# Autodesk Inventor assembly: mt32_case
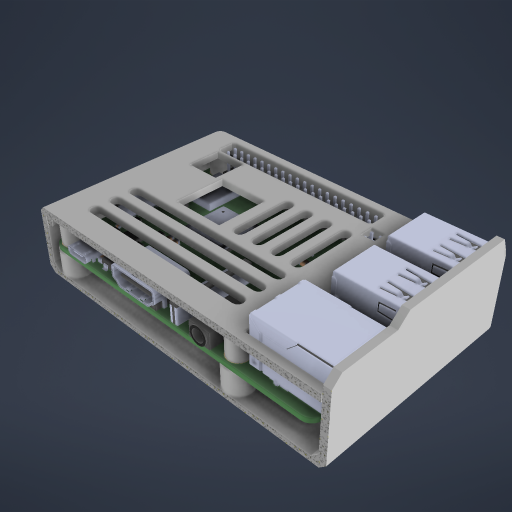
[picture p0: Inventor's stored thumbnail of the model, 512x512]
Saved by Autodesk Inventor 2024 (Build 280153000, 153)
## iProperties
Created: 2023-05-01
Part Number: mt32_case
Document SubType Name: Assembly
Designer: ancher
Author: ancher
## Documents named in this file (5)
- E:\RC\print_3d\mister\mt32_case\mt32_case.iam
- E:\RC\print_3d\mister\mt32_case\raspberry_pi3_b.ipt
- E:\RC\print_3d\mister\mt32_case\case_bottom.ipt
- E:\RC\print_3d\mister\mt32_case\case_top.ipt
- E:\RC\print_3d\mister\mt32_case\raspberry_pi3_b_.ipt
## Components (4 placed, 4 different names)
1. raspberry_pi3_b:1 — Mate:4, Mate:5, Mate:6, Mate:7, Mate:9
2. raspberry_pi3_b+:1 — Mate:10, Mate:11, Mate:12
3. case_bottom:1 — Mate:4, Mate:5, Mate:6, Mate:8, Mate:10, Mate:11, Mate:12
4. case_top:1 — Mate:7, Mate:8, Mate:9
## Relationships (9: Mate 9)
- Mate:4: raspberry_pi3_b:1 ↔ case_bottom:1
- Mate:5: raspberry_pi3_b:1 ↔ case_bottom:1
- Mate:6: raspberry_pi3_b:1 ↔ case_bottom:1
- Mate:7: raspberry_pi3_b:1 ↔ case_top:1
- Mate:8: case_bottom:1 ↔ case_top:1
- Mate:9: raspberry_pi3_b:1 ↔ case_top:1
- Mate:10: raspberry_pi3_b+:1 ↔ case_bottom:1
- Mate:11: raspberry_pi3_b+:1 ↔ case_bottom:1
- Mate:12: raspberry_pi3_b+:1 ↔ case_bottom:1
